# Autodesk Inventor assembly: front-mechanizm_MIR
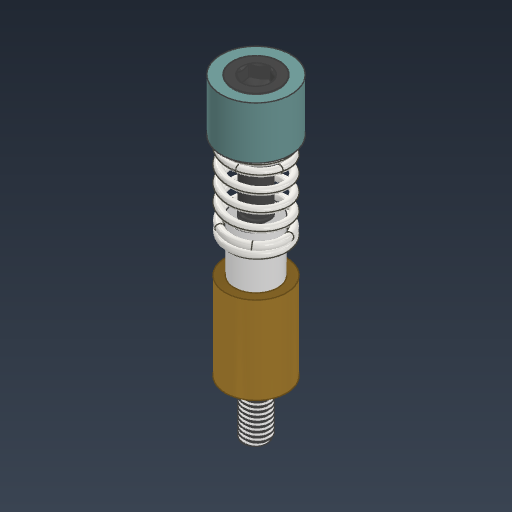
[picture p0: Inventor's stored thumbnail of the model, 512x512]
Saved by Autodesk Inventor 2023 (Build 270158000, 158)
## iProperties
Created: 2025-03-30
Part Number: front-mechanizm_MIR
Document SubType Name: Assembly
Designer: szymo
Mass: 6 g
Surface Area: 11.6592 cm^2
Volume: 0.501097 cm^3
Author: szymo
## Documents named in this file (6)
- D:\tech\robotyka\robots\evangelion\inventor-project\front-mechanizm_MIR.iam
- D:\tech\robotyka\robots\evangelion\inventor-project\rod_MIR.ipt
- D:\tech\robotyka\robots\evangelion\inventor-project\Compress Spring11_MIR.ipt
- D:\tech\robotyka\robots\evangelion\inventor-project\lozysko sf-1_MIR.ipt
- D:\tech\robotyka\robots\evangelion\inventor-project\rozszerzenie-m3_MIR.ipt
- D:\tech\robotyka\robots\evangelion\inventor-project\screws\m3x20M3_MIR.ipt
## Components (6 placed, 5 different names)
1. rod_MIR:1 — Mate:4, Flush:1, Mate:8, Mate:12, Mate:16, Mate:15
2. Compress Spring11_MIR:1 — Mate:4, Mate:11
3. lozysko sf-1_MIR:1 — Flush:1, Mate:8, Flush:18
4. rozszerzenie-m3_MIR:1 — Flush:18, Mate:11, Mate:14, Mate:13
5. m3x20M3_MIR:1 — Mate:14, Mate:13, Mate:12
6. m3x20M3_MIR:2 — Mate:16, Mate:15
## Relationships (10: Mate 8, Flush 2)
- Mate:4: rod_MIR:1 ↔ Compress Spring11_MIR:1
- Flush:1: rod_MIR:1 ↔ lozysko sf-1_MIR:1
- Mate:8: rod_MIR:1 ↔ lozysko sf-1_MIR:1
- Flush:18 (-20 mm): lozysko sf-1_MIR:1 ↔ rozszerzenie-m3_MIR:1
- Mate:11: Compress Spring11_MIR:1 ↔ rozszerzenie-m3_MIR:1
- Mate:14: rozszerzenie-m3_MIR:1 ↔ m3x20M3_MIR:1
- Mate:13: rozszerzenie-m3_MIR:1 ↔ m3x20M3_MIR:1
- Mate:12: rod_MIR:1 ↔ m3x20M3_MIR:1
- Mate:16: rod_MIR:1 ↔ m3x20M3_MIR:2
- Mate:15: rod_MIR:1 ↔ m3x20M3_MIR:2
